# Autodesk Inventor assembly: ABD_4mm_set
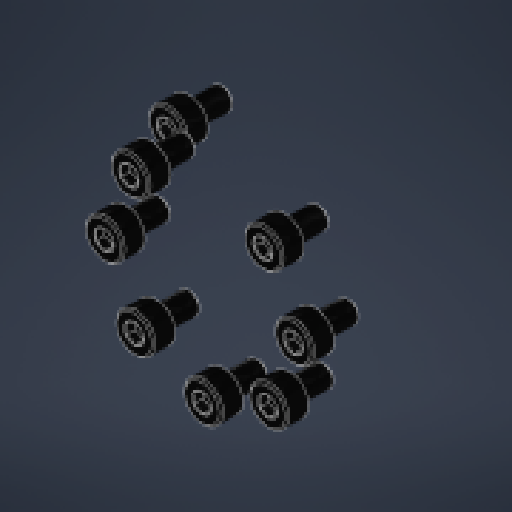
[picture p0: Inventor's stored thumbnail of the model, 512x512]
Saved by Autodesk Inventor 2024 (Build 280153000, 153)
## iProperties
Created: 2024-01-28
Part Number: ABD_4mm_set
Document SubType Name: Assembly
Designer: 김대겸
Author: 김대겸
## Documents named in this file (2)
- C:\Users\김대겸\Desktop\2024_Robit_Hardware\ROBOCUP_2024_eindhoven\부품\Bolt_Washer_Nut\ABD_4mm_set.iam
- C:\Users\김대겸\Desktop\2024_Robit_Hardware\ROBOCUP_2024_eindhoven\부품\Bolt_Washer_Nut\CSH-ST-M2_5-4_203.ipt
## Components (8 placed, 1 different names)
1. CSH-ST-M2_5-4_203:1
2. CSH-ST-M2_5-4_203:2
3. CSH-ST-M2_5-4_203:3
4. CSH-ST-M2_5-4_203:4
5. CSH-ST-M2_5-4_203:5
6. CSH-ST-M2_5-4_203:6
7. CSH-ST-M2_5-4_203:7
8. CSH-ST-M2_5-4_203:8
## Relationships (1: Flush 1)
- [Flush]: CSH-ST-M2_5-4_203:1 ↔ CSH-ST-M2_5-4_203:8
